# Autodesk Inventor assembly: BOTTOM ASSEMBLY BOX
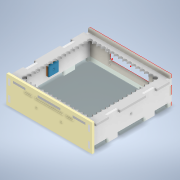
[picture p0: Inventor's stored thumbnail of the model, 180x180]
Saved by Autodesk Inventor 2022.3 (Build 263350030, 350C)
## iProperties
Created: 2021-06-17
Part Number: BOTTOM ASSEMBLY BOX
Document SubType Name: Assembly
Designer: benka
Author: benka
## Documents named in this file (10)
- C:\Users\Ben\OneDrive\Documents\GitHub\OpenMPD_Hardware\Cases\1x1 middle pillars\Model\BOTTOM ASSEMBLY BOX.iam
- C:\Users\Ben\OneDrive\Documents\GitHub\OpenMPD_Hardware\Cases\1x1 middle pillars\Model\ipt\NewBoardHolder.ipt
- C:\Users\Ben\OneDrive\Documents\GitHub\OpenMPD_Hardware\Cases\1x1 middle pillars\Model\ipt\case bottom sides.ipt
- C:\Users\Ben\OneDrive\Documents\GitHub\OpenMPD_Hardware\Cases\1x1 middle pillars\Model\ipt\board cover.ipt
- C:\Users\Ben\OneDrive\Documents\GitHub\OpenMPD_Hardware\Cases\1x1 middle pillars\Model\ipt\case bottom front.ipt
- C:\Users\Ben\OneDrive\Documents\GitHub\OpenMPD_Hardware\Cases\1x1 middle pillars\Model\ipt\case bottom back.ipt
- C:\Users\Ben\OneDrive\Documents\GitHub\OpenMPD_Hardware\Cases\1x1 middle pillars\Model\ipt\big holder.ipt
- C:\Users\Ben\OneDrive\Documents\GitHub\OpenMPD_Hardware\Cases\1x1 middle pillars\Model\ipt\big hex.ipt
- C:\Users\Ben\OneDrive\Documents\GitHub\OpenMPD_Hardware\Cases\1x1 middle pillars\Model\ipt\M4 Nut.ipt
- C:\Users\Ben\OneDrive\Documents\GitHub\OpenMPD_Hardware\Cases\1x1 middle pillars\Model\ipt\M2 Nut.ipt
## Components (22 placed, 9 different names)
1. NewBoardHolder:1 — Mate:81, Mate:82, Mate:83, Mate:84, Mate:85, Mate:86, Mate:87, Mate:88, Mate:89, Mate:92
2. case bottom sides:1 — Mate:87, Mate:88, Mate:89, Insert:12, Angle:2
3. case bottom sides:2 — Mate:84, Mate:85, Mate:86, Insert:11, Angle:1, Mate:107, Mate:109, Mate:110
4. board cover:1 — Mate:107, Mate:108, Mate:109, Mate:110
5. case bottom front:1 — Mate:92, Insert:9, Insert:10, Angle:3, Angle:4
6. case bottom back:1 — Mate:81, Mate:82, Mate:83, Mate:108
7. big hex:3 — Mate:96, Flush:5, Flush:6, Angle:3
8. M4 Nut:3 — Insert:5, Insert:10
9. M2 Nut:1
10. M2 Nut:2
11. M2 Nut:3
12. M2 Nut:4
13. big holder:5 — Mate:96, Flush:5, Flush:6, Insert:5
14. big hex:4 — Angle:1
15. M4 Nut:4 — Insert:11
16. big holder:6
17. big hex:5
18. M4 Nut:5 — Insert:12
19. big holder:7 — Angle:2
20. big hex:6 — Angle:4
21. M4 Nut:6 — Insert:9
22. big holder:8
## Relationships (38: Mate 18, Flush 8, Insert 8, Angle 4)
- Mate:81: NewBoardHolder:1 ↔ case bottom back:1
- Mate:82: NewBoardHolder:1 ↔ case bottom back:1
- Mate:83: NewBoardHolder:1 ↔ case bottom back:1
- Mate:84: NewBoardHolder:1 ↔ case bottom sides:2
- Mate:85: NewBoardHolder:1 ↔ case bottom sides:2
- Mate:86: NewBoardHolder:1 ↔ case bottom sides:2
- Mate:87: NewBoardHolder:1 ↔ case bottom sides:1
- Mate:88: NewBoardHolder:1 ↔ case bottom sides:1
- Mate:89: NewBoardHolder:1 ↔ case bottom sides:1
- Mate:92: NewBoardHolder:1 ↔ case bottom front:1
- Mate:96: big hex:3 ↔ big holder:5
- Flush:5: big hex:3 ↔ big holder:5
- Flush:6: big hex:3 ↔ big holder:5
- Insert:5: M4 Nut:3 ↔ big holder:5
- [Mate]: big hex:4 ↔ big holder:6
- [Flush]: big hex:4 ↔ big holder:6
- [Flush]: big hex:4 ↔ big holder:6
- [Insert]: M4 Nut:4 ↔ big holder:6
- [Mate]: big hex:5 ↔ big holder:7
- [Flush]: big hex:5 ↔ big holder:7
- [Flush]: big hex:5 ↔ big holder:7
- [Insert]: M4 Nut:5 ↔ big holder:7
- [Mate]: big hex:6 ↔ big holder:8
- [Flush]: big hex:6 ↔ big holder:8
- [Flush]: big hex:6 ↔ big holder:8
- [Insert]: M4 Nut:6 ↔ big holder:8
- Insert:9: case bottom front:1 ↔ M4 Nut:6
- Insert:10: case bottom front:1 ↔ M4 Nut:3
- Insert:11: case bottom sides:2 ↔ M4 Nut:4
- Insert:12: case bottom sides:1 ↔ M4 Nut:5
- Angle:1 (0 deg): case bottom sides:2 ↔ big hex:4
- Angle:2 (0 deg): case bottom sides:1 ↔ big holder:7
- Angle:3 (0 deg): case bottom front:1 ↔ big hex:3
- Angle:4 (0 deg): case bottom front:1 ↔ big hex:6
- Mate:107: case bottom sides:2 ↔ board cover:1
- Mate:108: board cover:1 ↔ case bottom back:1
- Mate:109: case bottom sides:2 ↔ board cover:1
- Mate:110: case bottom sides:2 ↔ board cover:1
## Named parameters: d153_d148 = 0 mm, d154_d149 = 0 mm, d155_d150 = 0 mm, d156_d152 = 0 mm, d157_d148 = 0 mm, d158_d149 = 0 mm, d159_d150 = 0 mm, d160_d152 = 0 mm, d161_d148 = 0 mm, d162_d149 = 0 mm, d163_d150 = 0 mm, d164_d152 = 0 mm
